# Autodesk Inventor assembly: moving-field-assm
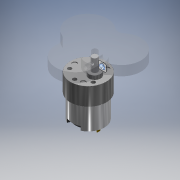
[picture p0: Inventor's stored thumbnail of the model, 180x180]
Saved by Autodesk Inventor 2017 (Build 210142000, 142)
## iProperties
Created: 2017-03-05
Part Number: moving-field-assm
Document SubType Name: Assembly
Designer: John
Author: John
## Documents named in this file (3)
- C:\Users\John\Dropbox\ECE115\pinball-project\moving-field-assm.iam
- C:\Users\John\Dropbox\ECE115\pinball-project\field-mover.ipt
- C:\Users\John\Dropbox\ECE115\geared_DC_Motor.ipt
## Components (2 placed, 2 different names)
1. field-mover:1 — Cylindrical:1
2. geared_DC_Motor:1 — Cylindrical:1
## Relationships (1: CylindricalJoint 1)
- Cylindrical:1: field-mover:1 ↔ geared_DC_Motor:1
